# Autodesk Inventor assembly: interface
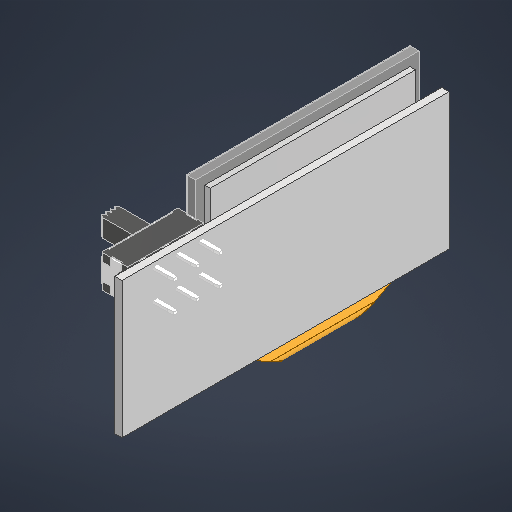
[picture p0: Inventor's stored thumbnail of the model, 512x512]
Saved by Autodesk Inventor 2026.2 (Build 302298000, 298)
## iProperties
Created: 2026-03-25
Part Number: interface
Document SubType Name: Assembly
Designer: szymo
Author: szymo
## Documents named in this file (5)
- C:\Users\szymo\Downloads\evangelion-turbo\inventor-project\interface.iam
- C:\Users\szymo\Downloads\evangelion-turbo\inventor-project\0.96 oled\0.96 oled\0.96 oled.ipt
- C:\Users\szymo\Downloads\evangelion-turbo\inventor-project\microswitch_EG1271A\microswitch_EG1271A\microswitch_EG1271A.ipt
- C:\Users\szymo\Downloads\evangelion-turbo\inventor-project\THMU 13 (SMD JOYSTICK)\THMU 13 (SMD JOYSTICK)\THMU 13 (SMD JOYSTICK).ipt
- C:\Users\szymo\Downloads\evangelion-turbo\inventor-project\interface-pcb.ipt
## Components (4 placed, 4 different names)
1. interface-pcb:1 — Mate:1, Mate:2, Flush:2, Mate:3, Mate:4, Mate:5, Flush:3, Mate:6
2. THMU 13 (SMD JOYSTICK):1 — Mate:4
3. microswitch_EG1271A:1 — Mate:5
4. 0.96 oled:1 — Flush:3, Mate:6
## Relationships (8: Mate 6, Flush 2)
- Mate:1: interface-pcb:1
- Mate:2: interface-pcb:1
- Flush:2: interface-pcb:1
- Mate:3: interface-pcb:1
- Mate:4: interface-pcb:1 ↔ THMU 13 (SMD JOYSTICK):1
- Mate:5: interface-pcb:1 ↔ microswitch_EG1271A:1
- Flush:3: interface-pcb:1 ↔ 0.96 oled:1
- Mate:6 (1.901 mm): interface-pcb:1 ↔ 0.96 oled:1
